# Autodesk Inventor assembly: GBX-901.1-grobox-casing
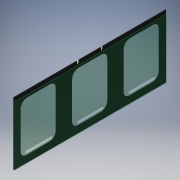
[picture p0: Inventor's stored thumbnail of the model, 180x180]
Saved by Autodesk Inventor 2019 (Build 230136000, 136)
## iProperties
Created: 2019-08-15
Part Number: GBX-901.1-grobox-casing
Document SubType Name: Assembly
Designer: Rene
Author: Rene
## Documents named in this file (5)
- C:\dev\c-scape\hardponics\dwg\grobox\GBX-901.1-grobox-casing.iam
- C:\dev\c-scape\hardponics\dwg\grobox\GBX-900.1-grobox-casing.iam
- C:\dev\c-scape\hardponics\dwg\eb_flow\EBF_910.1-eb-flow.iam
- C:\dev\c-scape\hardponics\dwg\grobox\GBX_020.1-front-MDF.ipt
- C:\dev\c-scape\hardponics\dwg\grobox\GBX_021.1-front-PMMA.ipt
## Components (6 placed, 4 different names)
1. GBX-900.1-grobox-casing:1 [sub-assembly] — Mate:1, Insert:1, Insert:2, Mate:2, Angle:1, Mate:3
2. GBX_020.1-front-MDF:1 — Mate:2, Angle:1, Mate:3, Mate:4, Mate:5, Mate:6, Flush:1
3. GBX_021.1-front-PMMA:1 — Mate:4, Mate:5, Mate:6, Flush:1
4. EBF_910.1-eb-flow:1 [sub-assembly] — Mate:1, Insert:1, Insert:2
5. EBF_910.1-eb-flow:2 [sub-assembly]
6. EBF_910.1-eb-flow:3 [sub-assembly]
## Component patterns: (3 elements, first: EBF_910.1-eb-flow:1)
## Relationships (10: Mate 6, Insert 2, Angle 1, Flush 1)
- Mate:1: GBX-900.1-grobox-casing:1 ↔ EBF_910.1-eb-flow:1
- Insert:1: GBX-900.1-grobox-casing:1 ↔ EBF_910.1-eb-flow:1
- Insert:2: GBX-900.1-grobox-casing:1 ↔ EBF_910.1-eb-flow:1
- Mate:2: GBX-900.1-grobox-casing:1 ↔ GBX_020.1-front-MDF:1
- Angle:1 (0 deg): GBX-900.1-grobox-casing:1 ↔ GBX_020.1-front-MDF:1
- Mate:3: GBX-900.1-grobox-casing:1 ↔ GBX_020.1-front-MDF:1
- Mate:4: GBX_020.1-front-MDF:1 ↔ GBX_021.1-front-PMMA:1
- Mate:5: GBX_020.1-front-MDF:1 ↔ GBX_021.1-front-PMMA:1
- Mate:6: GBX_020.1-front-MDF:1 ↔ GBX_021.1-front-PMMA:1
- Flush:1: GBX_020.1-front-MDF:1 ↔ GBX_021.1-front-PMMA:1
